# Autodesk Inventor assembly: 頭
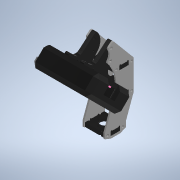
[picture p0: Inventor's stored thumbnail of the model, 180x180]
Saved by Autodesk Inventor 2020.4 (Build 244396000, 396)
## iProperties
Created: 2021-09-05
Part Number: 頭
Document SubType Name: Assembly
Designer: Masato
Author: Masato
## Documents named in this file (8)
- C:\Users\Masato\Documents\Inventor\CIT Brains_Inventor\OpenPlatform_ver3_0\上半身\頭\頭.iam
- C:\Users\Masato\Documents\Inventor\CIT Brains_Inventor\OpenPlatform_ver3_0\上半身\頭\KBCR-S02MU.ipt
- C:\Users\Masato\Documents\Inventor\CIT Brains_Inventor\OpenPlatform_ver3_0\上半身\頭\カメラ_メインフレーム.ipt
- C:\Users\Masato\Documents\Inventor\CIT Brains_Inventor\OpenPlatform_ver3_0\上半身\頭\カメラ_メインフレーム1_KBCR-S02MU.ipt
- C:\Users\Masato\Documents\Inventor\CIT Brains_Inventor\OpenPlatform_ver3_0\上半身\頭\カメラ_外装.ipt
- C:\Users\Masato\Documents\Inventor\CIT Brains_Inventor\OpenPlatform_ver3_0\上半身\頭\頭_サーボホーンフレーム.ipt
- C:\Users\Masato\Documents\Inventor\CIT Brains_Inventor\OpenPlatform_ver3_0\上半身\頭\頭_サブフレーム.ipt
- C:\Users\Masato\Documents\Inventor\CIT Brains_Inventor\OpenPlatform_ver3_0\上半身\頭\頭_メインフレーム.ipt
## Components (10 placed, 7 different names)
1. KBCR-S02MU:1 — 挿入:23, 挿入:24, 挿入:25, 挿入:26
2. カメラ_メインフレーム:1 — 挿入:3, 挿入:4, 挿入:7, 挿入:8
3. カメラ_メインフレーム:2 — 挿入:5, 挿入:6, 挿入:9, 挿入:10
4. カメラ_メインフレーム1_KBCR-S02MU:1 — 挿入:3, 挿入:4, 挿入:5, 挿入:6, 挿入:23, 挿入:24, 挿入:25, 挿入:26, 挿入:27, 挿入:28
5. カメラ_外装:1 — 挿入:27, 挿入:28
6. 頭_サーボホーンフレーム:1 — 挿入:29, 挿入:30, 挿入:31, 挿入:32
7. 頭_サブフレーム:1 — 挿入:11, 挿入:12, 挿入:15, 挿入:16
8. 頭_サブフレーム:2 — 挿入:13, 挿入:14, 挿入:17, 挿入:18
9. 頭_メインフレーム:1 — 挿入:7, 挿入:8, 挿入:11, 挿入:12, 挿入:13, 挿入:14, 挿入:29, 挿入:30
10. 頭_メインフレーム:2 — 挿入:9, 挿入:10, 挿入:15, 挿入:16, 挿入:17, 挿入:18, 挿入:31, 挿入:32
## Relationships (26: Insert 26)
- 挿入:3 [Insert]: カメラ_メインフレーム:1 ↔ カメラ_メインフレーム1_KBCR-S02MU:1
- 挿入:4 [Insert]: カメラ_メインフレーム:1 ↔ カメラ_メインフレーム1_KBCR-S02MU:1
- 挿入:5 [Insert]: カメラ_メインフレーム:2 ↔ カメラ_メインフレーム1_KBCR-S02MU:1
- 挿入:6 [Insert]: カメラ_メインフレーム:2 ↔ カメラ_メインフレーム1_KBCR-S02MU:1
- 挿入:7 [Insert]: カメラ_メインフレーム:1 ↔ 頭_メインフレーム:1
- 挿入:8 [Insert]: カメラ_メインフレーム:1 ↔ 頭_メインフレーム:1
- 挿入:9 [Insert]: カメラ_メインフレーム:2 ↔ 頭_メインフレーム:2
- 挿入:10 [Insert]: カメラ_メインフレーム:2 ↔ 頭_メインフレーム:2
- 挿入:11 [Insert]: 頭_サブフレーム:1 ↔ 頭_メインフレーム:1
- 挿入:12 [Insert]: 頭_サブフレーム:1 ↔ 頭_メインフレーム:1
- 挿入:13 [Insert]: 頭_サブフレーム:2 ↔ 頭_メインフレーム:1
- 挿入:14 [Insert]: 頭_サブフレーム:2 ↔ 頭_メインフレーム:1
- 挿入:15 [Insert]: 頭_サブフレーム:1 ↔ 頭_メインフレーム:2
- 挿入:16 [Insert]: 頭_サブフレーム:1 ↔ 頭_メインフレーム:2
- 挿入:17 [Insert]: 頭_サブフレーム:2 ↔ 頭_メインフレーム:2
- 挿入:18 [Insert]: 頭_サブフレーム:2 ↔ 頭_メインフレーム:2
- 挿入:23 [Insert]: KBCR-S02MU:1 ↔ カメラ_メインフレーム1_KBCR-S02MU:1
- 挿入:24 [Insert]: KBCR-S02MU:1 ↔ カメラ_メインフレーム1_KBCR-S02MU:1
- 挿入:25 [Insert]: KBCR-S02MU:1 ↔ カメラ_メインフレーム1_KBCR-S02MU:1
- 挿入:26 [Insert]: KBCR-S02MU:1 ↔ カメラ_メインフレーム1_KBCR-S02MU:1
- 挿入:27 [Insert]: カメラ_メインフレーム1_KBCR-S02MU:1 ↔ カメラ_外装:1
- 挿入:28 [Insert]: カメラ_メインフレーム1_KBCR-S02MU:1 ↔ カメラ_外装:1
- 挿入:29 [Insert]: 頭_サーボホーンフレーム:1 ↔ 頭_メインフレーム:1
- 挿入:30 [Insert]: 頭_サーボホーンフレーム:1 ↔ 頭_メインフレーム:1
- 挿入:31 [Insert]: 頭_サーボホーンフレーム:1 ↔ 頭_メインフレーム:2
- 挿入:32 [Insert]: 頭_サーボホーンフレーム:1 ↔ 頭_メインフレーム:2
